# Autodesk Inventor assembly: Ensamblaje1
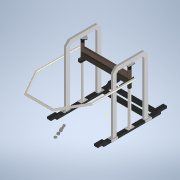
[picture p0: Inventor's stored thumbnail of the model, 180x180]
Saved by Autodesk Inventor 2021 (Build 250183000, 183)
## iProperties
Created: 2022-01-26
Part Number: Ensamblaje1
Document SubType Name: Conjunto soldado
Designer: arthu
Weld Material: Hierro, fundido
Author: arthu
## Documents named in this file (11)
- C:\Users\arthu\OneDrive\Escritorio\Maquina_ladrillo\Ponedora\Ensamblaje1.iam
- C:\Users\arthu\OneDrive\Escritorio\Maquina_ladrillo\Ponedora\Base.ipt
- C:\Users\arthu\OneDrive\Escritorio\Maquina_ladrillo\Ponedora\LateralD.ipt
- C:\Users\arthu\OneDrive\Escritorio\Maquina_ladrillo\Ponedora\union_ruedas.ipt
- C:\Users\arthu\OneDrive\Escritorio\Maquina_ladrillo\Ponedora\barra_palanca.ipt
- C:\Users\arthu\OneDrive\Documents\Inventor\Content Center Files\R2021\es-ES\SKF NUP\SKF NUPNUP 304 EC.ipt
- C:\Users\arthu\OneDrive\Documents\Inventor\Content Center Files\R2021\es-ES\GB_T 276-94 60000-2RS and 2LS\Bearing 6304-2LS GB_T 276-94.ipt
- C:\Users\arthu\OneDrive\Escritorio\Maquina_ladrillo\Ponedora\encaje.ipt
- C:\Users\arthu\OneDrive\Escritorio\Maquina_ladrillo\Ponedora\bocina1.ipt
- C:\Users\arthu\OneDrive\Escritorio\Maquina_ladrillo\Ponedora\bocina2.ipt
- C:\Users\arthu\OneDrive\Escritorio\Maquina_ladrillo\Ponedora\tubo_principal.ipt
## Components (22 placed, 10 different names)
1. Base:1 — Plana:1, Plana:2, Corredera:1, Corredera:2, Corredera:3, Corredera:4
2. LateralD:1 — Plana:1, De rotación:1
3. LateralD:2 — Plana:2, De rotación:2
4. union_ruedas:1 — Corredera:1
5. union_ruedas:2 — Corredera:2
6. union_ruedas:3 — Corredera:3
7. union_ruedas:4 — Corredera:4
8. barra_palanca:1
9. SKF NUP SKF NUPNUP 304 EC:1
10. SKF NUP SKF NUPNUP 304 EC:2
11. SKF NUP SKF NUPNUP 304 EC:3
12. SKF NUP SKF NUPNUP 304 EC:4
13. Rolling bearing GB/T 276-1994 Type 60000-2RS and 2LS 6304-2LS:1
14. Rolling bearing GB/T 276-1994 Type 60000-2RS and 2LS 6304-2LS:2
15. Rolling bearing GB/T 276-1994 Type 60000-2RS and 2LS 6304-2LS:3
16. Rolling bearing GB/T 276-1994 Type 60000-2RS and 2LS 6304-2LS:4
17. encaje:1 — De rotación:1, De rotación:3
18. encaje:2 — De rotación:2, Cilíndrica:1
19. bocina1:1 — Cilíndrica:1, De rotación:3, Cilíndrica:2
20. bocina2:1 — Cilíndrica:2
21. tubo_principal:1
22. tubo_principal:2
## Relationships (11: TranslationJoint 4, RevoluteJoint 3, PlanarJoint 2, CylindricalJoint 2)
- Plana:1: Base:1 ↔ LateralD:1
- Plana:2: Base:1 ↔ LateralD:2
- Corredera:1 [TranslationJoint]: Base:1 ↔ union_ruedas:1
- Corredera:2 [TranslationJoint]: Base:1 ↔ union_ruedas:2
- Corredera:3 [TranslationJoint]: Base:1 ↔ union_ruedas:3
- Corredera:4 [TranslationJoint]: Base:1 ↔ union_ruedas:4
- De rotación:1 [RevoluteJoint]: LateralD:1 ↔ encaje:1
- De rotación:2 [RevoluteJoint]: LateralD:2 ↔ encaje:2
- Cilíndrica:1 [CylindricalJoint]: encaje:2 ↔ bocina1:1
- De rotación:3 [RevoluteJoint]: encaje:1 ↔ bocina1:1
- Cilíndrica:2 [CylindricalJoint]: bocina1:1 ↔ bocina2:1
